# Autodesk Inventor assembly: szuflada150x400mm
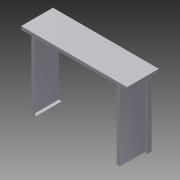
[picture p0: Inventor's stored thumbnail of the model, 180x180]
Saved by Autodesk Inventor 2013 (Build 170138000, 138)
## iProperties
Created: 2014-05-20
Part Number: szuflada150x400mm
Document SubType Name: Assembly
Designer: Piotr
Author: Piotr
## Documents named in this file (4)
- E:\3d_printer\szafka\szuflada150x400mm.iam
- E:\3d_printer\szafka\front szuflady 150mm.ipt
- E:\3d_printer\szafka\bok szuflady metalbox 150x400mm lewy.ipt
- E:\3d_printer\szafka\bok szuflady metalbox 150x400mm prawy.ipt
## Components (3 placed, 3 different names)
1. front szuflady 150mm:1 — Wstaw:1, Wstaw:2, Wstaw:3, Wstaw:4
2. bok szuflady metalbox 150x400mm lewy:1 — Wstaw:2, Wstaw:4
3. bok szuflady metalbox 150x400mm prawy:1 — Wstaw:1, Wstaw:3
## Relationships (4: Insert 4)
- Wstaw:1 [Insert]: front szuflady 150mm:1 ↔ bok szuflady metalbox 150x400mm prawy:1
- Wstaw:2 [Insert]: front szuflady 150mm:1 ↔ bok szuflady metalbox 150x400mm lewy:1
- Wstaw:3 [Insert]: front szuflady 150mm:1 ↔ bok szuflady metalbox 150x400mm prawy:1
- Wstaw:4 [Insert]: front szuflady 150mm:1 ↔ bok szuflady metalbox 150x400mm lewy:1
